# Autodesk Inventor assembly: 2f2
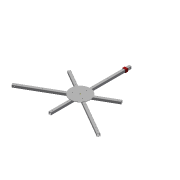
[picture p0: Inventor's stored thumbnail of the model, 180x180]
Saved by Autodesk Inventor 2017 (Build 210142000, 142)
## iProperties
Company: HERA Project
Created: 2013-06-27
Part Number: 2f2
Document SubType Name: Assembly
Designer: David DeBoer
Description: Feed backplane support assembly
Author: David DeBoer
Title: Feed backplane support
## Documents named in this file (6)
- C:\Users\krosie\Google Drive\HERA\hera-cad\feed\bpMechSupAssembly.iam
- C:\Users\krosie\Google Drive\HERA\hera-cad\feed\bpSupCross.ipt
- C:\Users\krosie\Google Drive\HERA\hera-cad\feed\bpSupInner1.ipt
- C:\Users\krosie\Google Drive\HERA\hera-cad\feed\bpPlate.ipt
- C:\Users\krosie\Google Drive\HERA\hera-cad\feed\bpSupInner2.ipt
- C:\Users\krosie\Google Drive\HERA\hera-cad\feed\squareNorthBand.ipt
## Components (7 placed, 5 different names)
1. bpSupCross:1 — Insert:2, Mate:5, Mate:7, Insert:7, Mate:9, Mate:10, Flush:1
2. bpSupInner1:2 — Insert:6, Mate:6
3. bpSupInner1:3 — Insert:5, Mate:8
4. bpPlate:1 — Insert:2, Mate:1, Mate:4, Insert:5, Insert:6, Insert:7
5. bpSupInner2:1 — Mate:1, Mate:7, Mate:8
6. bpSupInner2:2 — Mate:4, Mate:5, Mate:6
7. squareNorthBand:1 — Mate:9, Mate:10, Flush:1
## Relationships (13: Mate 8, Insert 4, Flush 1)
- Insert:2: bpSupCross:1 ↔ bpPlate:1
- Mate:1: bpPlate:1 ↔ bpSupInner2:1
- Mate:4: bpPlate:1 ↔ bpSupInner2:2
- Insert:5: bpSupInner1:3 ↔ bpPlate:1
- Insert:6: bpSupInner1:2 ↔ bpPlate:1
- Mate:5: bpSupCross:1 ↔ bpSupInner2:2
- Mate:6: bpSupInner1:2 ↔ bpSupInner2:2
- Mate:7: bpSupCross:1 ↔ bpSupInner2:1
- Mate:8: bpSupInner1:3 ↔ bpSupInner2:1
- Insert:7: bpSupCross:1 ↔ bpPlate:1
- Mate:9: bpSupCross:1 ↔ squareNorthBand:1
- Mate:10: bpSupCross:1 ↔ squareNorthBand:1
- Flush:1 (-38.1 mm): bpSupCross:1 ↔ squareNorthBand:1
